# Autodesk Inventor assembly: SSCSP12-10_MIR2
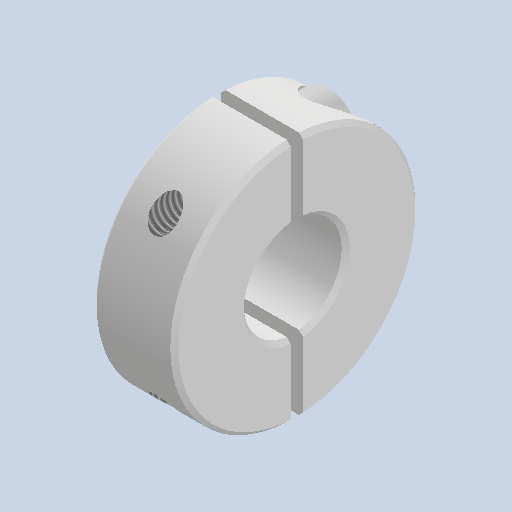
[picture p0: Inventor's stored thumbnail of the model, 512x512]
Saved by Autodesk Inventor 2025.2 (Build 292293000, 293)
## iProperties
Category: PARTsolutions
Company: MISUMI
Created: 2023-12-05
Part Number: SSCSP12-10_MIR2
Catalog Web Link: www.cadenas.de
Description: SCSP, PSCSP, SSCSP, SCNPA, SCNPAW-Set Collars - Separate - Standard Type
Vendor: MISUMI
Document SubType Name: Assembly
Designer: haruy
Manufacturer: MISUMI
Mass: 5.37187 g
Surface Area: 37.9033 cm^2
Volume: 5.37187 cm^3
Density: 1 g/cm^3
Title: SSCSP12-10
Author: Cadenas PARTsolutions
Comments: Set Collars - Separate - Standard Type
PSOL_IDENT_0: {$CADENAS_DATA/23d-libs/misumi/metric/03_set_collars/pscsp_asmtab.prj},212 {VTYP=3D},{STYP=ASSTAB},{
PSOL_IDENT_1: NB=SSCSP12-10},{LINA=SSCSP12-10},{NN=SCSP, PSCSP, SSCSP, SCNPA, SCNPAW},{DATE=18.06.2021 05:30:27},{
PSOL_IDENT_2: GEOMDATE=08.06.2021 03:00:18},{VERSION=},{LINEID=70},{WBVAR=MAT,ST,BS},{WBNUMERIC=BS}  {NB=SSCSP12-1
PSOL_IDENT_3: 0},{LINA=SSCSP12-10},{KT=DUMMY},{PN=SSCSP12-10},{TYPE=SSCSP},{TS=S},{MAT=304},{ST=-},{AC=Hexagon Soc
PSOL_IDENT_4: ket Head Cap Screws 2 Pcs. (SUS) },{D=12},{BS=10},{B1=8,10,12,15},{B2=8,10,12},{BALG=8,10,12,15},{D1=
PSOL_IDENT_5: 30},{M=M4},{THMD=4},{ST0= '-','-' },{DD=4.5},{R=3.75},{W=1.5},{X=10.0},{Y=5.0},{M1=M4},{M1A=M4},{P1=
PSOL_IDENT_6: 22.0},{P11=22},{C=0.5},{L=12},{MATA=  '1045','1045 Carbon Steel','304','304 Stainless Steel','2017','
PSOL_IDENT_7: 2017 Aluminum'   },{THMD1=4},{N=5.5},{N1=5.5},{P22=21.0},{P2=21.0},{PPATH=scsp_templ.prj}
NB: SSCSP12-10
NN: SCSP, PSCSP, SSCSP, SCNPA, SCNPAW
NT: Set Collars - Separate - Standard Type
NBSYN: $PN.
LINA: SSCSP12-10
CATALOG: Misumi
PN: SSCSP12-10
MAT: 304 Stainless Steel
ST: -
AC: Hexagon Socket Head Cap Screws 2 Pcs. (SUS)
D: 12
BS: 10
D1: 30
M: M4
DD: 4.5
R: 3.75
W: 1.5
X: 10
Y: 5
SUPPLIER: MISUMI
ARTICLENO: SSCSP12-10
BOMINFO: SSCSP12-10
CREATOR: CADENAS GmbH
## Documents named in this file (4)
- C:\Users\haruy\Documents\ロボコン\NHK2025\cad\nagahisa\base_weel\takagi_weel\Workspaces\作業スペース\takagi\omuni_wheel_ver3.0\parts\frequently used parts\セットカラー\SSCSP12-10\SSCSP12-10_MIR2.iam
- C:\Users\haruy\Documents\ロボコン\NHK2025\cad\nagahisa\base_weel\takagi_weel\Workspaces\作業スペース\takagi\omuni_wheel_ver3.0\parts\frequently used parts\セットカラー\SSCSP12-10\SSCSP12-10b_MIR2.ipt
- C:\Users\haruy\Documents\ロボコン\NHK2025\cad\nagahisa\base_weel\takagi_weel\Workspaces\作業スペース\takagi\omuni_wheel_ver3.0\parts\frequently used parts\セットカラー\SSCSP12-10\Slotted head cap screw ISO 4762 - M4x12_MIR2.ipt
- C:\Users\haruy\Documents\ロボコン\NHK2025\cad\nagahisa\base_weel\takagi_weel\Workspaces\作業スペース\takagi\omuni_wheel_ver3.0\parts\frequently used parts\セットカラー\SSCSP12-10\SSCSP12-10p_MIR2.ipt
## Components (4 placed, 3 different names)
1. SSCSP12-10b_MIR2:1 — body_screw_Z@1 <-> IP1_Z@2, body_screw2_Z@1 <-> IP1_Z@3, 1_2_Z@1 <-> 2_1_Z@4, 1_2_YZ@1 <-> 2_1_YZ@4
2. Slotted head cap screw ISO 4762 - M4x12_MIR2:1 — body_screw_Z@1 <-> IP1_Z@2
3. Slotted head cap screw ISO 4762 - M4x12_MIR2:2 — body_screw2_Z@1 <-> IP1_Z@3
4. SSCSP12-10p_MIR2:1 — 1_2_Z@1 <-> 2_1_Z@4, 1_2_YZ@1 <-> 2_1_YZ@4
## Relationships (4: Mate 3, Angle 1)
- body_screw_Z@1 <-> IP1_Z@2 [Mate]: SSCSP12-10b_MIR2:1 ↔ Slotted head cap screw ISO 4762 - M4x12_MIR2:1
- body_screw2_Z@1 <-> IP1_Z@3 [Mate]: SSCSP12-10b_MIR2:1 ↔ Slotted head cap screw ISO 4762 - M4x12_MIR2:2
- 1_2_Z@1 <-> 2_1_Z@4 [Mate]: SSCSP12-10b_MIR2:1 ↔ SSCSP12-10p_MIR2:1
- 1_2_YZ@1 <-> 2_1_YZ@4 [Angle] (0 deg): SSCSP12-10b_MIR2:1 ↔ SSCSP12-10p_MIR2:1
